# Autodesk Inventor assembly: assy-box
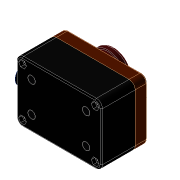
[picture p0: Inventor's stored thumbnail of the model, 180x180]
Saved by Autodesk Inventor 2022 (Build 260153000, 153)
## iProperties
Created: 2021-04-30
Part Number: assy-box
Document SubType Name: Assembly
Designer: yuta0
Author: yuta0
## Documents named in this file (10)
- C:\Users\yuta0\Documents\GitHub\catchrobo_hardware\emergency_switch_box\assy-box.iam
- C:\Users\yuta0\Documents\GitHub\catchrobo_hardware\emergency_switch_box\box.ipt
- C:\Users\yuta0\Documents\GitHub\catchrobo_hardware\emergency_switch_box\A165E_S_02.iam
- C:\Users\yuta0\Documents\GitHub\catchrobo_hardware\emergency_switch_box\box_top.ipt
- C:\Users\yuta0\Documents\GitHub\catchrobo_hardware\emergency_switch_box\box_bottom.ipt
- C:\Users\yuta0\Documents\GitHub\catchrobo_hardware\emergency_switch_box\LBNR3.ipt
- C:\Users\yuta0\Documents\GitHub\catchrobo_hardware\assy-robot\PLT-164-R-R.ipt
- C:\Users\yuta0\Documents\GitHub\catchrobo_hardware\assy-robot\holder_magnet.ipt
- C:\Users\yuta0\Documents\GitHub\catchrobo_hardware\emergency_switch_box\AP6MS54G.ipt
- C:\Users\yuta0\Documents\GitHub\catchrobo_hardware\assy-robot\CB3-35.ipt
## Components (18 placed, 9 different names)
1. box:1 — メイト:1, 角度:1, メイト:2
2. A165E_S_02:1 [sub-assembly] — メイト:1, 角度:1, メイト:2
3. box_top:1 — メイト:6, メイト:7, メイト:12, メイト:13
4. box_bottom:1 — メイト:3, メイト:5, メイト:8, メイト:9, メイト:10, フラッシュ:1, メイト:14
5. PLT-164-R-R:1 — メイト:8, メイト:9, メイト:10
6. AP6MS54G:1 — メイト:12, メイト:13
7. CB3-35:1 — メイト:6, メイト:7
8. LBNR3:1 — メイト:3, メイト:5
9. CB3-35:2
10. LBNR3:2
11. CB3-35:3
12. LBNR3:3
13. CB3-35:4
14. LBNR3:4
15. holder_magnet:1 — フラッシュ:1, メイト:14
16. holder_magnet:2
17. holder_magnet:3
18. holder_magnet:4
## Component patterns: (4 elements, first: CB3-35:1 + LBNR3:1), (4 elements, first: holder_magnet:1)
## Relationships (14: Mate 12, Angle 1, Flush 1)
- メイト:1 [Mate]: box:1 ↔ A165E_S_02:1
- 角度:1 [Angle] (0 deg): box:1 ↔ A165E_S_02:1
- メイト:2 [Mate]: box:1 ↔ A165E_S_02:1
- メイト:3 [Mate]: box_bottom:1 ↔ LBNR3:1
- メイト:5 [Mate]: box_bottom:1 ↔ LBNR3:1
- メイト:6 [Mate]: box_top:1 ↔ CB3-35:1
- メイト:7 [Mate]: box_top:1 ↔ CB3-35:1
- メイト:8 [Mate]: box_bottom:1 ↔ PLT-164-R-R:1
- メイト:9 [Mate]: box_bottom:1 ↔ PLT-164-R-R:1
- メイト:10 [Mate]: box_bottom:1 ↔ PLT-164-R-R:1
- フラッシュ:1 [Flush]: box_bottom:1 ↔ holder_magnet:1
- メイト:12 [Mate]: box_top:1 ↔ AP6MS54G:1
- メイト:13 [Mate]: box_top:1 ↔ AP6MS54G:1
- メイト:14 [Mate]: box_bottom:1 ↔ holder_magnet:1
